# Autodesk Inventor assembly: 全体
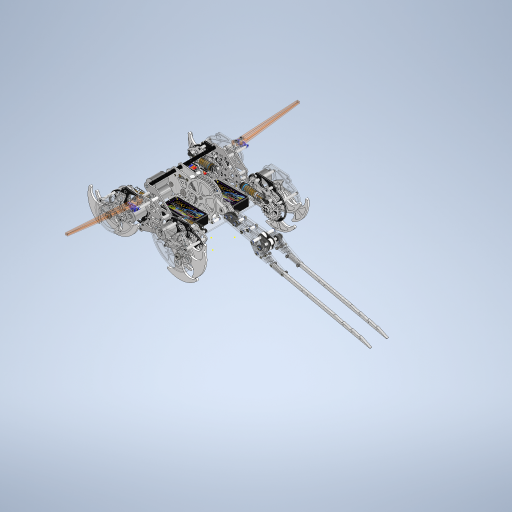
[picture p0: Inventor's stored thumbnail of the model, 512x512]
Saved by Autodesk Inventor 2023 (Build 270158030, 158C)
## iProperties
Created: 2022-05-13
Part Number: 全体
Document SubType Name: Assembly
Designer: muzho
Mass: 3276.34 g
Surface Area: 9316.07 cm^2
Volume: 1317.68 cm^3
Density: 2.48645 g/cm^3
Author: muzho
## Documents named in this file (9)
- C:\Users\muzho\Documents\srdc\srdc_2\全体.iam
- C:\Users\muzho\Documents\srdc\srdc_2\脚\足全体.iam
- C:\Users\muzho\Documents\srdc\srdc_2\バッテリー BAKUSO.ipt
- C:\Users\muzho\Documents\srdc\srdc_2\MC402CR.ipt
- C:\Users\muzho\Documents\srdc\srdc_2\脚\シャフト.ipt
- C:\Users\muzho\Documents\srdc\srdc_2\下板.ipt
- C:\Users\muzho\Documents\srdc\srdc_2\脚\足全体_反対.iam
- C:\Users\muzho\Documents\srdc\srdc_2\ねじ\M4皿ネジ　8.ipt
- C:\Users\muzho\Documents\srdc\srdc_2\アーム\アームアセンブリ.iam
## Components (12 placed, 8 different names)
1. バッテリー BAKUSO:1 — フラッシュ:4, メイト:4
2. バッテリー BAKUSO:2 — メイト:7, メイト:19
3. MC402CR:1 — メイト:8
4. MC402CR:2 — メイト:9, メイト:20
5. MC402CR:3 — フラッシュ:4, メイト:10, メイト:20
6. シャフト:1 — 挿入:1, 挿入:2, メイト:18
7. 下板:1 — メイト:4, メイト:7, メイト:8, メイト:9, メイト:10, フラッシュ:5, フラッシュ:6, メイト:15, メイト:16, メイト:17, メイト:19
8. 足全体:1 [sub-assembly] — 挿入:1, フラッシュ:5, 挿入:4, メイト:16
9. 足全体_反対:1 [sub-assembly] — フラッシュ:6, 挿入:2, 挿入:3, メイト:17
10. M4皿ネジ　8:1 — 挿入:4
11. M4皿ネジ　8:2 — 挿入:3
12. アームアセンブリ:1 [sub-assembly] — メイト:15, メイト:18
## Relationships (18: Mate 11, Insert 4, Flush 3)
- フラッシュ:4 [Flush]: バッテリー BAKUSO:1 ↔ MC402CR:3
- メイト:4 [Mate]: バッテリー BAKUSO:1 ↔ 下板:1
- メイト:7 [Mate]: バッテリー BAKUSO:2 ↔ 下板:1
- メイト:8 [Mate]: MC402CR:1 ↔ 下板:1
- メイト:9 [Mate]: MC402CR:2 ↔ 下板:1
- メイト:10 [Mate]: MC402CR:3 ↔ 下板:1
- 挿入:1 [Insert]: シャフト:1 ↔ 足全体:1
- フラッシュ:5 [Flush]: 下板:1 ↔ 足全体:1
- フラッシュ:6 [Flush]: 下板:1 ↔ 足全体_反対:1
- 挿入:2 [Insert]: シャフト:1 ↔ 足全体_反対:1
- 挿入:3 [Insert]: 足全体_反対:1 ↔ M4皿ネジ　8:2
- 挿入:4 [Insert]: 足全体:1 ↔ M4皿ネジ　8:1
- メイト:15 [Mate]: 下板:1 ↔ アームアセンブリ:1
- メイト:16 [Mate]: 下板:1 ↔ 足全体:1
- メイト:17 [Mate]: 下板:1 ↔ 足全体_反対:1
- メイト:18 [Mate]: シャフト:1 ↔ アームアセンブリ:1
- メイト:19 [Mate]: バッテリー BAKUSO:2 ↔ 下板:1
- メイト:20 [Mate] (2 mm): MC402CR:2 ↔ MC402CR:3
